# Autodesk Inventor assembly: Tetrix Honors Robotics
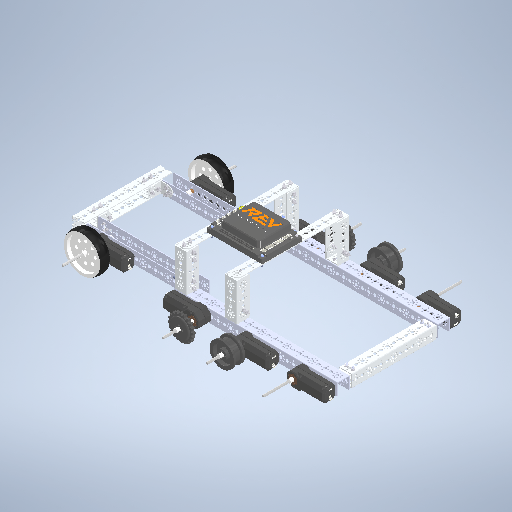
[picture p0: Inventor's stored thumbnail of the model, 512x512]
Saved by Autodesk Inventor 2025 (Build 290162010, 162A)
## iProperties
Created: 2024-11-13
Part Number: Tetrix Honors Robotics
Document SubType Name: Assembly
Designer: William Alexander
Author: William Alexander
## Documents named in this file (24)
- C:\Users\wa229389\Documents\William Alexander\Vehicles\Tetrix Honors Robotics.iam
- C:\Users\wa229389\Documents\William Alexander\Tetrix SW Parts(2)\Tetrix 416mm Channel(2)\Tetrix 416mm Channel(2).ipt
- C:\Users\wa229389\Documents\William Alexander\Tetrix SW Parts(2)\Tetrix Tank Tread Idler Wheel(2)\Tetrix Tank Tread Idler Wheel(2).ipt
- C:\Users\wa229389\Documents\William Alexander\Tetrix SW Parts(2)\Tetrix Screw 6-32 x 0.5(2)\Tetrix Screw 6-32 x 0.5(2).ipt
- C:\Users\wa229389\Documents\William Alexander\Tetrix SW Parts(2)\Tetrix Flat 288mm x26mm(2)\Tetrix Flat 288mm x26mm(2).ipt
- C:\Users\wa229389\Documents\William Alexander\Tetrix SW Parts(2)\Tetrix 96mm Channel(2)\Tetrix 96mm Channel(2).ipt
- C:\Users\wa229389\Documents\William Alexander\Tetrix SW Parts(2)\Tetrix L Bracket(2)\Tetrix L Bracket(2).ipt
- C:\Users\wa229389\Documents\William Alexander\Tetrix SW Parts(2)\Tetrix Inside C Connectors(2)\Tetrix Inside C Connectors(2).ipt
- C:\Users\wa229389\Documents\William Alexander\Tetrix SW Parts(2)\Tetrix Kep Nut(2)\Tetrix Kep Nut(2).ipt
- C:\Users\wa229389\Documents\William Alexander\Tetrix SW Parts(2)\Tetrix Tank Tread Sprocket(2)\Tetrix Tank Tread Sprocket(2).ipt
- C:\Users\wa229389\Documents\William Alexander\Tetrix SW Parts\Tetrix 416mm Channel\Tetrix 416mm Channel.ipt
- C:\Users\wa229389\Documents\William Alexander\Tetrix SW Parts\Tetrix Kep Nut\Tetrix Kep Nut.ipt
- C:\Users\wa229389\Documents\William Alexander\Tetrix SW Parts\Tetrix Screw 6-32 x 0.5\Tetrix Screw 6-32 x 0.5.ipt
- C:\Users\wa229389\Documents\William Alexander\Tetrix SW Parts\Tetrix 416mm Channel - Copy\Tetrix 416mm Channel - Copy.ipt
- C:\Users\wa229389\Documents\William Alexander\tetrix-part-library-inventor-2018-files-1.snapshot.27\Fasteners\Socket Head Cap Screws\32mm Socket Head Cap Screw.ipt
- C:\Users\wa229389\Documents\William Alexander\Tetrix SW Parts(2)\Tetrix 416mm Channel(2) - Copy\Tetrix 416mm Channel(2) - Copy.ipt
- C:\Users\wa229389\Documents\William Alexander\tetrix-part-library-inventor-2018-files-1.snapshot.27\Fasteners\Kep Nut.ipt
- C:\Users\wa229389\Documents\William Alexander\Tetrix SW Parts(2)\Tetrix Axle Spacer 0.375(2)\Tetrix Axle Spacer 0.375(2).ipt
- C:\Users\wa229389\Documents\William Alexander\rev-core-hex-motor-1.snapshot.2\REV-41-1300 (1)\REV-41-1300 (1).ipt
- C:\Users\wa229389\Documents\William Alexander\rev-core-hex-motor-1.snapshot.2\REV-41-1347\REV-41-1347.ipt
- C:\Users\wa229389\Documents\William Alexander\Tetrix SW Parts(2)\Tetrix 4 inch Wheel(2)\Tetrix 4 inch Wheel(2).ipt
- C:\Users\wa229389\Documents\William Alexander\Tetrix SW Parts(2)\Tetrix 4.7mm x 4mm L Bronze Bushing(2)\Tetrix 4.7mm x 4mm L Bronze Bushing(2).ipt
- C:\Users\wa229389\Documents\William Alexander\Tetrix SW Parts\Tetrix Ball Head Cap Screw 6-32 x 0.375\Tetrix Ball Head Cap Screw 6-32 x 0.375.ipt
- C:\Users\wa229389\Documents\William Alexander\tetrix-part-library-inventor-2018-files-1.snapshot.27\REV Expansion Hub.ipt
## Components (249 placed, 23 different names)
1. Tetrix Tank Tread Idler Wheel(2):1 — Insert:188, Insert:265
2. Tetrix Tank Tread Idler Wheel(2):2 — Insert:187, Insert:260
3. Tetrix Screw 6-32 x 0.5(2):1 — Insert:34
4. Tetrix Screw 6-32 x 0.5(2):2 — Insert:33
5. Tetrix Screw 6-32 x 0.5(2):3 — Insert:32
6. Tetrix Screw 6-32 x 0.5(2):4 — Insert:35
7. Tetrix Flat 288mm x26mm(2):1 — Mate:12, Insert:106, Insert:107, Insert:289, Mate:21, Mate:22
8. Tetrix Flat 288mm x26mm(2):2 — Mate:14, Insert:103, Insert:108, Insert:111, Insert:112, Mate:18, Insert:288
9. Tetrix 96mm Channel(2):1 — Mate:10, Insert:53, Insert:68, Insert:69, Insert:70, Insert:86, Insert:87, Insert:178
10. Tetrix 96mm Channel(2):2 — Mate:11, Insert:55, Insert:66, Insert:67, Insert:72, Insert:73, Insert:83, Insert:84, Insert:85
11. Tetrix L Bracket(2):1 — Insert:97, Mate:15, Insert:135, Insert:136, Insert:143, Insert:144, Insert:148
12. Tetrix L Bracket(2):2 — Insert:96, Insert:137, Insert:138, Insert:141, Insert:142, Insert:145, Insert:146, Insert:150
13. Tetrix Inside C Connectors(2):2 — Mate:2, Insert:2, Insert:3, Insert:4, Insert:5, Mate:6, Insert:16, Insert:17, Insert:18, Insert:19
14. Tetrix 416mm Channel(2):2 — Mate:2, Mate:3, Mate:4, Insert:6, Insert:7, Mate:5, Insert:12, Insert:13, Insert:14, Insert:15
15. Tetrix Kep Nut(2):3 — Insert:43
16. Tetrix Tank Tread Sprocket(2):1 — Insert:198, Insert:259
17. Tetrix Kep Nut(2):5 — Insert:41
18. Tetrix Kep Nut(2):6 — Insert:40
19. Tetrix Kep Nut(2):7 — Insert:42
20. Tetrix Screw 6-32 x 0.5(2):6 — Insert:3
21. Tetrix Screw 6-32 x 0.5(2):7 — Insert:2
22. Tetrix 416mm Channel:1 — Mate:6, Insert:20, Insert:21, Insert:22, Insert:23, Mate:8, Insert:32, Insert:33, Insert:34, Insert:35, Insert:52, Insert:98, Insert:202, Insert:205, Insert:211, Insert:213, Insert:215, Insert:230, Insert:231, Insert:233, Insert:276, Insert:277, Insert:278, Insert:279, Insert:280, Insert:281
23. Tetrix Kep Nut:1 — Insert:7
24. Tetrix Kep Nut:2 — Insert:6
25. Tetrix Kep Nut:3 — Mate:3
26. Tetrix Kep Nut:4 — Mate:4
27. Tetrix Screw 6-32 x 0.5:1 — Insert:5
28. Tetrix Screw 6-32 x 0.5:2 — Insert:4
29. Tetrix Screw 6-32 x 0.5:3 — Insert:9
30. Tetrix Screw 6-32 x 0.5:4 — Insert:10
31. Tetrix Screw 6-32 x 0.5:5 — Insert:11
32. Tetrix Screw 6-32 x 0.5:6 — Insert:8
33. Tetrix Inside C Connectors(2):3 — Mate:5, Insert:8, Insert:9, Insert:10, Insert:11, Mate:7, Insert:24, Insert:25, Insert:26, Insert:27
34. Tetrix Kep Nut(2):8 — Insert:15
35. Tetrix Kep Nut(2):9 — Insert:14
36. Tetrix Kep Nut(2):10 — Insert:13
37. Tetrix Kep Nut(2):11 — Insert:12
38. Tetrix Kep Nut(2):12 — Insert:22
39. Tetrix Kep Nut(2):13 — Insert:23
40. Tetrix Kep Nut(2):14 — Insert:20
41. Tetrix Kep Nut(2):15 — Insert:21
42. Tetrix 416mm Channel:2 — Mate:7, Insert:28, Insert:29, Insert:30, Insert:31, Mate:9, Insert:48, Insert:49, Insert:50, Insert:51, Insert:54, Insert:99, Insert:201, Insert:203, Insert:210, Insert:212, Insert:214, Insert:234, Insert:236, Insert:237, Insert:266, Insert:267, Insert:268, Insert:269, Insert:270, Insert:271
43. Tetrix Screw 6-32 x 0.5:7 — Insert:17
44. Tetrix Screw 6-32 x 0.5:8 — Insert:16
45. Tetrix Screw 6-32 x 0.5:9 — Insert:19
46. Tetrix Screw 6-32 x 0.5:10 — Insert:18
47. Tetrix Screw 6-32 x 0.5:11 — Insert:24
48. Tetrix Screw 6-32 x 0.5:12 — Insert:25
49. Tetrix Screw 6-32 x 0.5:13 — Insert:26
50. Tetrix Screw 6-32 x 0.5:14 — Insert:27
51. Tetrix Kep Nut:5 — Insert:29
52. Tetrix Kep Nut:6 — Insert:28
53. Tetrix Kep Nut:7 — Insert:31
54. Tetrix Kep Nut:8 — Insert:30
55. Tetrix 416mm Channel - Copy:1 — Mate:8, Insert:40, Insert:41, Insert:42, Insert:43, Insert:97, Insert:129, Insert:130, Insert:147, Insert:206, Insert:232, Insert:274, Insert:275
56. Tetrix 416mm Channel - Copy:2 — Mate:9, Insert:44, Insert:45, Insert:46, Insert:47, Insert:96, Insert:131, Insert:132, Insert:149, Insert:208, Insert:235, Insert:272, Insert:273
57. Tetrix Kep Nut:9 — Insert:45
58. Tetrix Kep Nut:10 — Insert:44
59. Tetrix Kep Nut:11 — Insert:47
60. Tetrix Kep Nut:12 — Insert:46
61. Tetrix Screw 6-32 x 0.5:15 — Insert:49
62. Tetrix Screw 6-32 x 0.5:16 — Insert:51
63. Tetrix Screw 6-32 x 0.5:17 — Insert:48
64. Tetrix Screw 6-32 x 0.5:18 — Insert:50
65. Tetrix Inside C Connectors(2):4 — Insert:53, Insert:58, Insert:60, Insert:61, Mate:19, Mate:20
66. Tetrix Inside C Connectors(2):5 — Insert:54, Mate:11, Insert:74, Insert:82, Insert:94, Insert:199
67. Tetrix Inside C Connectors(2):6 — Insert:55, Mate:12, Insert:62, Insert:63, Insert:64, Insert:65, Insert:104, Insert:105
68. Tetrix Inside C Connectors(2):7 — Insert:52, Mate:10, Insert:92, Insert:93, Insert:95, Insert:177
69. Tetrix Screw 6-32 x 0.5(2):8 — Insert:60
70. Tetrix Screw 6-32 x 0.5(2):11 — Insert:58
71. Tetrix Screw 6-32 x 0.5(2):12 — Insert:61
72. Tetrix Screw 6-32 x 0.5(2):13 — Insert:62
73. Tetrix Screw 6-32 x 0.5(2):15 — Insert:65
74. Tetrix Screw 6-32 x 0.5(2):16 — Insert:63
75. Tetrix Screw 6-32 x 0.5(2):17 — Insert:64
76. Tetrix Kep Nut(2):16 — Insert:66
77. Tetrix Kep Nut(2):17 — Insert:68
78. Tetrix Kep Nut(2):18 — Insert:69
79. Tetrix Kep Nut(2):19 — Insert:67
80. Tetrix Kep Nut(2):20 — Insert:72
81. Tetrix Kep Nut(2):21 — Insert:70
82. Tetrix Kep Nut(2):22 — Insert:73
83. Tetrix Kep Nut(2):24 — Insert:85
84. Tetrix Kep Nut(2):25 — Insert:87
85. Tetrix Kep Nut(2):26 — Insert:86
86. Tetrix Kep Nut(2):28 — Insert:83
87. Tetrix Kep Nut(2):29 — Insert:84
88. Tetrix Screw 6-32 x 0.5(2):25 — Insert:74
89. Tetrix Screw 6-32 x 0.5(2):31 — Insert:82
90. 32mm Socket Head Cap Screw:1 — Insert:92
91. 32mm Socket Head Cap Screw:2 — Insert:93
92. 32mm Socket Head Cap Screw:3 — Insert:94
93. Tetrix Screw 6-32 x 0.5(2):32 — Insert:95
94. Tetrix 96mm Channel(2):3 — Insert:101, Insert:102, Insert:171, Insert:172, Insert:185, Insert:186
95. Tetrix 96mm Channel(2):4 — Insert:100, Mate:13, Insert:175, Insert:176, Insert:181, Insert:182
96. Tetrix Inside C Connectors(2):9 — Insert:102, Insert:109, Insert:110
97. Tetrix Inside C Connectors(2):10 — Insert:99, Insert:100, Insert:173, Insert:174, Insert:179, Insert:180, Insert:200
98. Tetrix Inside C Connectors(2):11 — Insert:98, Insert:101, Insert:169, Insert:170, Insert:183, Insert:184, Insert:204
99. Tetrix Inside C Connectors(2):12 — Mate:13, Mate:14
100. Tetrix Screw 6-32 x 0.5(2):33 — Insert:103
101. Tetrix Screw 6-32 x 0.5(2):34 — Insert:105
102. Tetrix Screw 6-32 x 0.5(2):35 — Insert:104
103. Tetrix Kep Nut(2):32 — Insert:107
104. Tetrix Kep Nut(2):33 — Insert:106
105. Tetrix Kep Nut(2):34 — Insert:112
106. Tetrix Kep Nut(2):35 — Insert:111
107. Tetrix Screw 6-32 x 0.5(2):36 — Insert:109
108. Tetrix Screw 6-32 x 0.5(2):37 — Insert:110
109. Tetrix Screw 6-32 x 0.5(2):38 — Insert:108
110. Tetrix 416mm Channel(2) - Copy:1 — Insert:133, Insert:134, Mate:16, Mate:17, Insert:155, Insert:156
111. Tetrix Screw 6-32 x 0.5(2):39 — Insert:131
112. Tetrix Kep Nut(2):40 — Insert:143
113. Tetrix Kep Nut(2):41 — Insert:146
114. Tetrix Kep Nut(2):42 — Insert:144
115. Tetrix Kep Nut(2):43 — Insert:145
116. Tetrix Screw 6-32 x 0.5(2):44 — Insert:132
117. Tetrix Screw 6-32 x 0.5(2):45 — Insert:130
118. Tetrix Screw 6-32 x 0.5(2):46 — Insert:129
119. Tetrix Kep Nut(2):44 — Insert:150
120. Tetrix Kep Nut(2):45 — Mate:17
121. Tetrix Kep Nut(2):46 — Insert:138
122. Tetrix Kep Nut(2):47 — Mate:16
123. Tetrix Kep Nut(2):48 — Insert:137
124. Tetrix Kep Nut(2):49 — Insert:148
125. Tetrix Kep Nut(2):50 — Insert:136
126. Tetrix Kep Nut(2):51 — Insert:135
127. Tetrix Screw 6-32 x 0.5(2):47 — Insert:139
128. Tetrix Screw 6-32 x 0.5(2):48 — Insert:141
129. Tetrix Screw 6-32 x 0.5(2):49 — Insert:142
130. Tetrix Screw 6-32 x 0.5(2):50 — Insert:140
131. Tetrix Screw 6-32 x 0.5(2):51 — Insert:151
132. Tetrix Screw 6-32 x 0.5(2):52 — Insert:152
133. Tetrix Screw 6-32 x 0.5(2):53 — Insert:149
134. Tetrix Screw 6-32 x 0.5(2):54 — Insert:147
135. Tetrix Inside C Connectors(2):13 — Mate:15, Insert:133, Insert:139, Insert:140, Insert:151, Insert:152
136. Tetrix Inside C Connectors(2):14 — Insert:134, Insert:153, Insert:154
137. Tetrix Screw 6-32 x 0.5(2):55 — Insert:153
138. Tetrix Screw 6-32 x 0.5(2):56 — Insert:154
139. Tetrix Kep Nut(2):52 — Insert:156
140. Tetrix Kep Nut(2):53 — Insert:155
141. Tetrix Kep Nut(2):54 — Insert:176
142. Tetrix Kep Nut(2):55 — Insert:175
143. Tetrix Kep Nut(2):56 — Insert:182
144. Tetrix Kep Nut(2):57 — Insert:181
145. Tetrix Kep Nut(2):58 — Insert:172
146. Tetrix Kep Nut(2):59 — Insert:171
147. Tetrix Kep Nut(2):61 — Insert:178
148. Tetrix Screw 6-32 x 0.5(2):57 — Insert:170
149. Tetrix Screw 6-32 x 0.5(2):58 — Insert:169
150. Tetrix Screw 6-32 x 0.5(2):59 — Insert:174
151. Tetrix Screw 6-32 x 0.5(2):60 — Insert:173
152. Tetrix Screw 6-32 x 0.5(2):61 — Insert:184
153. Tetrix Screw 6-32 x 0.5(2):62 — Insert:183
154. Tetrix Screw 6-32 x 0.5(2):63 — Insert:180
155. Tetrix Screw 6-32 x 0.5(2):64 — Insert:179
156. 32mm Socket Head Cap Screw:4 — Insert:177
157. Tetrix Kep Nut(2):62 — Insert:185
158. Tetrix Kep Nut(2):63 — Insert:186
159. Tetrix Axle Spacer 0.375(2):2 — Insert:188
160. Tetrix Axle Spacer 0.375(2):3 — Insert:187
161. REV-41-1300 (1):1 — Insert:230, Insert:255
162. REV-41-1300 (1):2 — Insert:231, Insert:256
163. REV-41-1300 (1):3 — Insert:235, Insert:254
164. REV-41-1300 (1):4 — Insert:232, Insert:257
165. REV-41-1300 (1):5 — Insert:234, Insert:251
166. REV-41-1300 (1):6 — Insert:233, Insert:238
167. REV-41-1300 (1):7 — Insert:236, Insert:252
168. REV-41-1300 (1):8 — Insert:237, Insert:253
169. Tetrix Axle Spacer 0.375(2):7 — Insert:198, Insert:258
170. Tetrix Screw 6-32 x 0.5(2):65 — Insert:204
171. Tetrix Screw 6-32 x 0.5(2):66 — Insert:199
172. Tetrix Screw 6-32 x 0.5(2):67 — Insert:200
173. Tetrix Kep Nut(2):64 — Insert:205
174. Tetrix Kep Nut(2):65 — Insert:202
175. Tetrix Kep Nut(2):66 — Insert:203
176. Tetrix Kep Nut(2):67 — Insert:201
177. Tetrix 4 inch Wheel(2):1 — Insert:261, Insert:263
178. Tetrix 4 inch Wheel(2):2 — Insert:262, Insert:264
179. Tetrix 4.7mm x 4mm L Bronze Bushing(2):1 — Insert:215, Insert:219
180. Tetrix 4.7mm x 4mm L Bronze Bushing(2):2 — Insert:214, Insert:216
181. Tetrix 4.7mm x 4mm L Bronze Bushing(2):3 — Insert:213, Insert:220
182. Tetrix 4.7mm x 4mm L Bronze Bushing(2):4 — Insert:212, Insert:217
183. Tetrix 4.7mm x 4mm L Bronze Bushing(2):5 — Insert:211, Insert:221
184. Tetrix 4.7mm x 4mm L Bronze Bushing(2):6 — Insert:210, Insert:218
185. Tetrix 4.7mm x 4mm L Bronze Bushing(2):7 — Insert:208, Insert:209
186. Tetrix 4.7mm x 4mm L Bronze Bushing(2):8 — Insert:206, Insert:207
187. REV-41-1347:11 — Insert:225
188. REV-41-1347:12 — Insert:226
189. REV-41-1347:13 — Insert:228
190. REV-41-1347:14 — Insert:229
191. REV-41-1347:15 — Insert:227
192. REV-41-1347:16 — Insert:224
193. REV-41-1347:17 — Insert:223
194. REV-41-1347:18 — Insert:222
195. Tetrix Axle Spacer 0.375(2):8 — Insert:221, Insert:229
196. Tetrix Axle Spacer 0.375(2):9 — Insert:220, Insert:228
197. Tetrix Axle Spacer 0.375(2):10 — Insert:219, Insert:227
198. Tetrix Axle Spacer 0.375(2):11 — Insert:218, Insert:226
199. Tetrix Axle Spacer 0.375(2):12 — Insert:217, Insert:225
200. Tetrix Axle Spacer 0.375(2):13 — Insert:216, Insert:224
201. Tetrix Axle Spacer 0.375(2):14 — Insert:209, Insert:222
202. Tetrix Axle Spacer 0.375(2):15 — Insert:207, Insert:223
203. Tetrix Axle Spacer 0.375(2):16 — Insert:259
204. Tetrix Axle Spacer 0.375(2):17 — Insert:262
205. Tetrix Axle Spacer 0.375(2):18 — Insert:261
206. Tetrix Axle Spacer 0.375(2):19 — Insert:257, Insert:263
207. Tetrix Axle Spacer 0.375(2):20 — Insert:256, Insert:260
208. Tetrix Axle Spacer 0.375(2):21 — Insert:253
209. Tetrix Axle Spacer 0.375(2):23 — Insert:238, Insert:239
210. Tetrix Axle Spacer 0.375(2):24 — Insert:251, Insert:258
211. Tetrix Axle Spacer 0.375(2):25 — Insert:252, Insert:265
212. Tetrix Axle Spacer 0.375(2):26 — Insert:254, Insert:264
213. Tetrix Axle Spacer 0.375(2):27 — Insert:255
214. Tetrix Tank Tread Sprocket(2):3 — Insert:240, Insert:241, Insert:245, Insert:246, Insert:247, Insert:248, Insert:249, Insert:250
215. Tetrix Axle Spacer 0.375(2):32 — Insert:241
216. Tetrix Axle Spacer 0.375(2):33 — Insert:239, Insert:240
217. Kep Nut:7 — Insert:245
218. Kep Nut:8 — Insert:247
219. Kep Nut:9 — Insert:246
220. 32mm Socket Head Cap Screw:5 — Insert:248
221. 32mm Socket Head Cap Screw:6 — Insert:249
222. 32mm Socket Head Cap Screw:7 — Insert:250
223. Tetrix Ball Head Cap Screw 6-32 x 0.375:1 — Insert:267
224. Tetrix Ball Head Cap Screw 6-32 x 0.375:2 — Insert:266
225. Tetrix Ball Head Cap Screw 6-32 x 0.375:3 — Insert:268
226. Tetrix Ball Head Cap Screw 6-32 x 0.375:4 — Insert:269
227. Tetrix Ball Head Cap Screw 6-32 x 0.375:5 — Insert:270
228. Tetrix Ball Head Cap Screw 6-32 x 0.375:6 — Insert:271
229. Tetrix Ball Head Cap Screw 6-32 x 0.375:7 — Insert:273
230. Tetrix Ball Head Cap Screw 6-32 x 0.375:8 — Insert:272
231. Tetrix Ball Head Cap Screw 6-32 x 0.375:9 — Insert:277
232. Tetrix Ball Head Cap Screw 6-32 x 0.375:10 — Insert:276
233. Tetrix Ball Head Cap Screw 6-32 x 0.375:11 — Insert:275
234. Tetrix Ball Head Cap Screw 6-32 x 0.375:12 — Insert:274
235. Tetrix Ball Head Cap Screw 6-32 x 0.375:13 — Insert:278
236. Tetrix Ball Head Cap Screw 6-32 x 0.375:14 — Insert:279
237. Tetrix Ball Head Cap Screw 6-32 x 0.375:15 — Insert:281
238. Tetrix Ball Head Cap Screw 6-32 x 0.375:16 — Insert:280
239. REV Expansion Hub:1 — Insert:283, Insert:285, Mate:18, Insert:286, Insert:287
240. Tetrix Kep Nut(2):70 — Insert:288
241. Tetrix Kep Nut(2):71 — Insert:289
242. 32mm Socket Head Cap Screw:9 — Insert:285
243. 32mm Socket Head Cap Screw:10 — Insert:283
244. Tetrix Screw 6-32 x 0.5(2):68 — Insert:287
245. Tetrix Screw 6-32 x 0.5(2):69 — Insert:286
246. Tetrix Kep Nut(2):72 — Mate:21
247. Tetrix Kep Nut(2):73 — Mate:22
248. Tetrix Screw 6-32 x 0.5(2):70 — Mate:19
249. Tetrix Screw 6-32 x 0.5(2):71 — Mate:20
## Relationships (248: Insert 227, Mate 21)
- Mate:2: Tetrix Inside C Connectors(2):2 ↔ Tetrix 416mm Channel(2):2
- Insert:2: Tetrix Inside C Connectors(2):2 ↔ Tetrix Screw 6-32 x 0.5(2):7
- Insert:3: Tetrix Inside C Connectors(2):2 ↔ Tetrix Screw 6-32 x 0.5(2):6
- Mate:3: Tetrix 416mm Channel(2):2 ↔ Tetrix Kep Nut:3
- Mate:4: Tetrix 416mm Channel(2):2 ↔ Tetrix Kep Nut:4
- Insert:4: Tetrix Inside C Connectors(2):2 ↔ Tetrix Screw 6-32 x 0.5:2
- Insert:5: Tetrix Inside C Connectors(2):2 ↔ Tetrix Screw 6-32 x 0.5:1
- Insert:6: Tetrix 416mm Channel(2):2 ↔ Tetrix Kep Nut:2
- Insert:7: Tetrix 416mm Channel(2):2 ↔ Tetrix Kep Nut:1
- Mate:5: Tetrix 416mm Channel(2):2 ↔ Tetrix Inside C Connectors(2):3
- Insert:8: Tetrix Screw 6-32 x 0.5:6 ↔ Tetrix Inside C Connectors(2):3
- Insert:9: Tetrix Screw 6-32 x 0.5:3 ↔ Tetrix Inside C Connectors(2):3
- Insert:10: Tetrix Screw 6-32 x 0.5:4 ↔ Tetrix Inside C Connectors(2):3
- Insert:11: Tetrix Screw 6-32 x 0.5:5 ↔ Tetrix Inside C Connectors(2):3
- Insert:12: Tetrix 416mm Channel(2):2 ↔ Tetrix Kep Nut(2):11
- Insert:13: Tetrix 416mm Channel(2):2 ↔ Tetrix Kep Nut(2):10
- Insert:14: Tetrix 416mm Channel(2):2 ↔ Tetrix Kep Nut(2):9
- Insert:15: Tetrix 416mm Channel(2):2 ↔ Tetrix Kep Nut(2):8
- Mate:6: Tetrix Inside C Connectors(2):2 ↔ Tetrix 416mm Channel:1
- Mate:7: Tetrix Inside C Connectors(2):3 ↔ Tetrix 416mm Channel:2
- Insert:16: Tetrix Inside C Connectors(2):2 ↔ Tetrix Screw 6-32 x 0.5:8
- Insert:17: Tetrix Inside C Connectors(2):2 ↔ Tetrix Screw 6-32 x 0.5:7
- Insert:18: Tetrix Inside C Connectors(2):2 ↔ Tetrix Screw 6-32 x 0.5:10
- Insert:19: Tetrix Inside C Connectors(2):2 ↔ Tetrix Screw 6-32 x 0.5:9
- Insert:20: Tetrix 416mm Channel:1 ↔ Tetrix Kep Nut(2):14
- Insert:21: Tetrix 416mm Channel:1 ↔ Tetrix Kep Nut(2):15
- Insert:22: Tetrix 416mm Channel:1 ↔ Tetrix Kep Nut(2):12
- Insert:23: Tetrix 416mm Channel:1 ↔ Tetrix Kep Nut(2):13
- Insert:24: Tetrix Inside C Connectors(2):3 ↔ Tetrix Screw 6-32 x 0.5:11
- Insert:25: Tetrix Inside C Connectors(2):3 ↔ Tetrix Screw 6-32 x 0.5:12
- Insert:26: Tetrix Inside C Connectors(2):3 ↔ Tetrix Screw 6-32 x 0.5:13
- Insert:27: Tetrix Inside C Connectors(2):3 ↔ Tetrix Screw 6-32 x 0.5:14
- Insert:28: Tetrix 416mm Channel:2 ↔ Tetrix Kep Nut:6
- Insert:29: Tetrix 416mm Channel:2 ↔ Tetrix Kep Nut:5
- Insert:30: Tetrix 416mm Channel:2 ↔ Tetrix Kep Nut:8
- Insert:31: Tetrix 416mm Channel:2 ↔ Tetrix Kep Nut:7
- Mate:8: Tetrix 416mm Channel:1 ↔ Tetrix 416mm Channel - Copy:1
- Mate:9: Tetrix 416mm Channel:2 ↔ Tetrix 416mm Channel - Copy:2
- Insert:32: Tetrix Screw 6-32 x 0.5(2):3 ↔ Tetrix 416mm Channel:1
- Insert:33: Tetrix Screw 6-32 x 0.5(2):2 ↔ Tetrix 416mm Channel:1
- Insert:34: Tetrix Screw 6-32 x 0.5(2):1 ↔ Tetrix 416mm Channel:1
- Insert:35: Tetrix Screw 6-32 x 0.5(2):4 ↔ Tetrix 416mm Channel:1
- Insert:40: Tetrix Kep Nut(2):6 ↔ Tetrix 416mm Channel - Copy:1
- Insert:41: Tetrix Kep Nut(2):5 ↔ Tetrix 416mm Channel - Copy:1
- Insert:42: Tetrix Kep Nut(2):7 ↔ Tetrix 416mm Channel - Copy:1
- Insert:43: Tetrix Kep Nut(2):3 ↔ Tetrix 416mm Channel - Copy:1
- Insert:44: Tetrix 416mm Channel - Copy:2 ↔ Tetrix Kep Nut:10
- Insert:45: Tetrix 416mm Channel - Copy:2 ↔ Tetrix Kep Nut:9
- Insert:46: Tetrix 416mm Channel - Copy:2 ↔ Tetrix Kep Nut:12
- Insert:47: Tetrix 416mm Channel - Copy:2 ↔ Tetrix Kep Nut:11
- Insert:48: Tetrix 416mm Channel:2 ↔ Tetrix Screw 6-32 x 0.5:17
- Insert:49: Tetrix 416mm Channel:2 ↔ Tetrix Screw 6-32 x 0.5:15
- Insert:50: Tetrix 416mm Channel:2 ↔ Tetrix Screw 6-32 x 0.5:18
- Insert:51: Tetrix 416mm Channel:2 ↔ Tetrix Screw 6-32 x 0.5:16
- Insert:52: Tetrix 416mm Channel:1 ↔ Tetrix Inside C Connectors(2):7
- Mate:10: Tetrix 96mm Channel(2):1 ↔ Tetrix Inside C Connectors(2):7
- Insert:53: Tetrix 96mm Channel(2):1 ↔ Tetrix Inside C Connectors(2):4
- Insert:54: Tetrix 416mm Channel:2 ↔ Tetrix Inside C Connectors(2):5
- Mate:11: Tetrix 96mm Channel(2):2 ↔ Tetrix Inside C Connectors(2):5
- Insert:55: Tetrix 96mm Channel(2):2 ↔ Tetrix Inside C Connectors(2):6
- Mate:12: Tetrix Flat 288mm x26mm(2):1 ↔ Tetrix Inside C Connectors(2):6
- Insert:58: Tetrix Inside C Connectors(2):4 ↔ Tetrix Screw 6-32 x 0.5(2):11
- Insert:60: Tetrix Inside C Connectors(2):4 ↔ Tetrix Screw 6-32 x 0.5(2):8
- Insert:61: Tetrix Inside C Connectors(2):4 ↔ Tetrix Screw 6-32 x 0.5(2):12
- Insert:62: Tetrix Inside C Connectors(2):6 ↔ Tetrix Screw 6-32 x 0.5(2):13
- Insert:63: Tetrix Inside C Connectors(2):6 ↔ Tetrix Screw 6-32 x 0.5(2):16
- Insert:64: Tetrix Inside C Connectors(2):6 ↔ Tetrix Screw 6-32 x 0.5(2):17
- Insert:65: Tetrix Inside C Connectors(2):6 ↔ Tetrix Screw 6-32 x 0.5(2):15
- Insert:66: Tetrix 96mm Channel(2):2 ↔ Tetrix Kep Nut(2):16
- Insert:67: Tetrix 96mm Channel(2):2 ↔ Tetrix Kep Nut(2):19
- Insert:68: Tetrix 96mm Channel(2):1 ↔ Tetrix Kep Nut(2):17
- Insert:69: Tetrix 96mm Channel(2):1 ↔ Tetrix Kep Nut(2):18
- Insert:70: Tetrix 96mm Channel(2):1 ↔ Tetrix Kep Nut(2):21
- Insert:72: Tetrix 96mm Channel(2):2 ↔ Tetrix Kep Nut(2):20
- Insert:73: Tetrix 96mm Channel(2):2 ↔ Tetrix Kep Nut(2):22
- Insert:74: Tetrix Inside C Connectors(2):5 ↔ Tetrix Screw 6-32 x 0.5(2):25
- Insert:82: Tetrix Inside C Connectors(2):5 ↔ Tetrix Screw 6-32 x 0.5(2):31
- Insert:83: Tetrix 96mm Channel(2):2 ↔ Tetrix Kep Nut(2):28
- Insert:84: Tetrix 96mm Channel(2):2 ↔ Tetrix Kep Nut(2):29
- Insert:85: Tetrix 96mm Channel(2):2 ↔ Tetrix Kep Nut(2):24
- Insert:86: Tetrix 96mm Channel(2):1 ↔ Tetrix Kep Nut(2):26
- Insert:87: Tetrix 96mm Channel(2):1 ↔ Tetrix Kep Nut(2):25
- Insert:92: Tetrix Inside C Connectors(2):7 ↔ 32mm Socket Head Cap Screw:1
- Insert:93: Tetrix Inside C Connectors(2):7 ↔ 32mm Socket Head Cap Screw:2
- Insert:94: Tetrix Inside C Connectors(2):5 ↔ 32mm Socket Head Cap Screw:3
- Insert:95: Tetrix Inside C Connectors(2):7 ↔ Tetrix Screw 6-32 x 0.5(2):32
- Insert:96: Tetrix L Bracket(2):2 ↔ Tetrix 416mm Channel - Copy:2
- Insert:97: Tetrix L Bracket(2):1 ↔ Tetrix 416mm Channel - Copy:1
- Insert:98: Tetrix 416mm Channel:1 ↔ Tetrix Inside C Connectors(2):11
- Insert:99: Tetrix 416mm Channel:2 ↔ Tetrix Inside C Connectors(2):10
- Insert:100: Tetrix 96mm Channel(2):4 ↔ Tetrix Inside C Connectors(2):10
- Insert:101: Tetrix 96mm Channel(2):3 ↔ Tetrix Inside C Connectors(2):11
- Insert:102: Tetrix 96mm Channel(2):3 ↔ Tetrix Inside C Connectors(2):9
- Mate:13: Tetrix 96mm Channel(2):4 ↔ Tetrix Inside C Connectors(2):12
- Mate:14: Tetrix Flat 288mm x26mm(2):2 ↔ Tetrix Inside C Connectors(2):12
- Insert:103: Tetrix Flat 288mm x26mm(2):2 ↔ Tetrix Screw 6-32 x 0.5(2):33
- Insert:104: Tetrix Inside C Connectors(2):6 ↔ Tetrix Screw 6-32 x 0.5(2):35
- Insert:105: Tetrix Inside C Connectors(2):6 ↔ Tetrix Screw 6-32 x 0.5(2):34
- Insert:106: Tetrix Flat 288mm x26mm(2):1 ↔ Tetrix Kep Nut(2):33
- Insert:107: Tetrix Flat 288mm x26mm(2):1 ↔ Tetrix Kep Nut(2):32
- Insert:108: Tetrix Flat 288mm x26mm(2):2 ↔ Tetrix Screw 6-32 x 0.5(2):38
- Insert:109: Tetrix Inside C Connectors(2):9 ↔ Tetrix Screw 6-32 x 0.5(2):36
- Insert:110: Tetrix Inside C Connectors(2):9 ↔ Tetrix Screw 6-32 x 0.5(2):37
- Insert:111: Tetrix Flat 288mm x26mm(2):2 ↔ Tetrix Kep Nut(2):35
- Insert:112: Tetrix Flat 288mm x26mm(2):2 ↔ Tetrix Kep Nut(2):34
- Insert:129: Tetrix 416mm Channel - Copy:1 ↔ Tetrix Screw 6-32 x 0.5(2):46
- Insert:130: Tetrix 416mm Channel - Copy:1 ↔ Tetrix Screw 6-32 x 0.5(2):45
- Insert:131: Tetrix 416mm Channel - Copy:2 ↔ Tetrix Screw 6-32 x 0.5(2):39
- Insert:132: Tetrix 416mm Channel - Copy:2 ↔ Tetrix Screw 6-32 x 0.5(2):44
- Mate:15: Tetrix L Bracket(2):1 ↔ Tetrix Inside C Connectors(2):13
- Insert:133: Tetrix 416mm Channel(2) - Copy:1 ↔ Tetrix Inside C Connectors(2):13
- Insert:134: Tetrix 416mm Channel(2) - Copy:1 ↔ Tetrix Inside C Connectors(2):14
- Insert:135: Tetrix L Bracket(2):1 ↔ Tetrix Kep Nut(2):51
- Insert:136: Tetrix L Bracket(2):1 ↔ Tetrix Kep Nut(2):50
- Insert:137: Tetrix L Bracket(2):2 ↔ Tetrix Kep Nut(2):48
- Insert:138: Tetrix L Bracket(2):2 ↔ Tetrix Kep Nut(2):46
- Insert:139: Tetrix Screw 6-32 x 0.5(2):47 ↔ Tetrix Inside C Connectors(2):13
- Insert:140: Tetrix Screw 6-32 x 0.5(2):50 ↔ Tetrix Inside C Connectors(2):13
- Insert:141 (2.54 mm): Tetrix L Bracket(2):2 ↔ Tetrix Screw 6-32 x 0.5(2):48
- Insert:142 (2.54 mm): Tetrix L Bracket(2):2 ↔ Tetrix Screw 6-32 x 0.5(2):49
- Insert:143: Tetrix L Bracket(2):1 ↔ Tetrix Kep Nut(2):40
- Insert:144: Tetrix L Bracket(2):1 ↔ Tetrix Kep Nut(2):42
- Insert:145: Tetrix L Bracket(2):2 ↔ Tetrix Kep Nut(2):43
- Insert:146: Tetrix L Bracket(2):2 ↔ Tetrix Kep Nut(2):41
- Insert:147: Tetrix 416mm Channel - Copy:1 ↔ Tetrix Screw 6-32 x 0.5(2):54
- Insert:148: Tetrix L Bracket(2):1 ↔ Tetrix Kep Nut(2):49
- Insert:149: Tetrix 416mm Channel - Copy:2 ↔ Tetrix Screw 6-32 x 0.5(2):53
- Insert:150: Tetrix L Bracket(2):2 ↔ Tetrix Kep Nut(2):44
- Insert:151: Tetrix Screw 6-32 x 0.5(2):51 ↔ Tetrix Inside C Connectors(2):13
- Insert:152: Tetrix Screw 6-32 x 0.5(2):52 ↔ Tetrix Inside C Connectors(2):13
- Insert:153: Tetrix Inside C Connectors(2):14 ↔ Tetrix Screw 6-32 x 0.5(2):55
- Insert:154: Tetrix Inside C Connectors(2):14 ↔ Tetrix Screw 6-32 x 0.5(2):56
- Mate:16: Tetrix 416mm Channel(2) - Copy:1 ↔ Tetrix Kep Nut(2):47
- Mate:17: Tetrix 416mm Channel(2) - Copy:1 ↔ Tetrix Kep Nut(2):45
- Insert:155: Tetrix 416mm Channel(2) - Copy:1 ↔ Tetrix Kep Nut(2):53
- Insert:156: Tetrix 416mm Channel(2) - Copy:1 ↔ Tetrix Kep Nut(2):52
- Insert:169: Tetrix Inside C Connectors(2):11 ↔ Tetrix Screw 6-32 x 0.5(2):58
- Insert:170: Tetrix Inside C Connectors(2):11 ↔ Tetrix Screw 6-32 x 0.5(2):57
- Insert:171: Tetrix 96mm Channel(2):3 ↔ Tetrix Kep Nut(2):59
- Insert:172: Tetrix 96mm Channel(2):3 ↔ Tetrix Kep Nut(2):58
- Insert:173: Tetrix Inside C Connectors(2):10 ↔ Tetrix Screw 6-32 x 0.5(2):60
- Insert:174: Tetrix Inside C Connectors(2):10 ↔ Tetrix Screw 6-32 x 0.5(2):59
- Insert:175: Tetrix 96mm Channel(2):4 ↔ Tetrix Kep Nut(2):55
- Insert:176: Tetrix 96mm Channel(2):4 ↔ Tetrix Kep Nut(2):54
- Insert:177: Tetrix Inside C Connectors(2):7 ↔ 32mm Socket Head Cap Screw:4
- Insert:178: Tetrix 96mm Channel(2):1 ↔ Tetrix Kep Nut(2):61
- Insert:179: Tetrix Inside C Connectors(2):10 ↔ Tetrix Screw 6-32 x 0.5(2):64
- Insert:180: Tetrix Inside C Connectors(2):10 ↔ Tetrix Screw 6-32 x 0.5(2):63
- Insert:181: Tetrix 96mm Channel(2):4 ↔ Tetrix Kep Nut(2):57
- Insert:182: Tetrix 96mm Channel(2):4 ↔ Tetrix Kep Nut(2):56
- Insert:183: Tetrix Inside C Connectors(2):11 ↔ Tetrix Screw 6-32 x 0.5(2):62
- Insert:184: Tetrix Inside C Connectors(2):11 ↔ Tetrix Screw 6-32 x 0.5(2):61
- Insert:185: Tetrix 96mm Channel(2):3 ↔ Tetrix Kep Nut(2):62
- Insert:186: Tetrix 96mm Channel(2):3 ↔ Tetrix Kep Nut(2):63
- Insert:187: Tetrix Tank Tread Idler Wheel(2):2 ↔ Tetrix Axle Spacer 0.375(2):3
- Insert:188: Tetrix Tank Tread Idler Wheel(2):1 ↔ Tetrix Axle Spacer 0.375(2):2
- Insert:198: Tetrix Tank Tread Sprocket(2):1 ↔ Tetrix Axle Spacer 0.375(2):7
- Insert:199: Tetrix Inside C Connectors(2):5 ↔ Tetrix Screw 6-32 x 0.5(2):66
- Insert:200: Tetrix Inside C Connectors(2):10 ↔ Tetrix Screw 6-32 x 0.5(2):67
- Insert:201: Tetrix 416mm Channel:2 ↔ Tetrix Kep Nut(2):67
- Insert:202: Tetrix 416mm Channel:1 ↔ Tetrix Kep Nut(2):65
- Insert:203: Tetrix 416mm Channel:2 ↔ Tetrix Kep Nut(2):66
- Insert:204: Tetrix Inside C Connectors(2):11 ↔ Tetrix Screw 6-32 x 0.5(2):65
- Insert:205: Tetrix 416mm Channel:1 ↔ Tetrix Kep Nut(2):64
- Insert:206: Tetrix 416mm Channel - Copy:1 ↔ Tetrix 4.7mm x 4mm L Bronze Bushing(2):8
- Insert:207: Tetrix 4.7mm x 4mm L Bronze Bushing(2):8 ↔ Tetrix Axle Spacer 0.375(2):15
- Insert:208: Tetrix 416mm Channel - Copy:2 ↔ Tetrix 4.7mm x 4mm L Bronze Bushing(2):7
- Insert:209: Tetrix 4.7mm x 4mm L Bronze Bushing(2):7 ↔ Tetrix Axle Spacer 0.375(2):14
- Insert:210: Tetrix 416mm Channel:2 ↔ Tetrix 4.7mm x 4mm L Bronze Bushing(2):6
- Insert:211: Tetrix 416mm Channel:1 ↔ Tetrix 4.7mm x 4mm L Bronze Bushing(2):5
- Insert:212: Tetrix 416mm Channel:2 ↔ Tetrix 4.7mm x 4mm L Bronze Bushing(2):4
- Insert:213: Tetrix 416mm Channel:1 ↔ Tetrix 4.7mm x 4mm L Bronze Bushing(2):3
- Insert:214: Tetrix 416mm Channel:2 ↔ Tetrix 4.7mm x 4mm L Bronze Bushing(2):2
- Insert:215: Tetrix 416mm Channel:1 ↔ Tetrix 4.7mm x 4mm L Bronze Bushing(2):1
- Insert:216: Tetrix 4.7mm x 4mm L Bronze Bushing(2):2 ↔ Tetrix Axle Spacer 0.375(2):13
- Insert:217: Tetrix 4.7mm x 4mm L Bronze Bushing(2):4 ↔ Tetrix Axle Spacer 0.375(2):12
- Insert:218: Tetrix 4.7mm x 4mm L Bronze Bushing(2):6 ↔ Tetrix Axle Spacer 0.375(2):11
- Insert:219: Tetrix 4.7mm x 4mm L Bronze Bushing(2):1 ↔ Tetrix Axle Spacer 0.375(2):10
- Insert:220: Tetrix 4.7mm x 4mm L Bronze Bushing(2):3 ↔ Tetrix Axle Spacer 0.375(2):9
- Insert:221: Tetrix 4.7mm x 4mm L Bronze Bushing(2):5 ↔ Tetrix Axle Spacer 0.375(2):8
- Insert:222: REV-41-1347:18 ↔ Tetrix Axle Spacer 0.375(2):14
- Insert:223: REV-41-1347:17 ↔ Tetrix Axle Spacer 0.375(2):15
- Insert:224: REV-41-1347:16 ↔ Tetrix Axle Spacer 0.375(2):13
- Insert:225: REV-41-1347:11 ↔ Tetrix Axle Spacer 0.375(2):12
- Insert:226: REV-41-1347:12 ↔ Tetrix Axle Spacer 0.375(2):11
- Insert:227: REV-41-1347:15 ↔ Tetrix Axle Spacer 0.375(2):10
- Insert:228: REV-41-1347:13 ↔ Tetrix Axle Spacer 0.375(2):9
- Insert:229: REV-41-1347:14 ↔ Tetrix Axle Spacer 0.375(2):8
- Insert:230: Tetrix 416mm Channel:1 ↔ REV-41-1300 (1):1
- Insert:231: Tetrix 416mm Channel:1 ↔ REV-41-1300 (1):2
- Insert:232: Tetrix 416mm Channel - Copy:1 ↔ REV-41-1300 (1):4
- Insert:233: Tetrix 416mm Channel:1 ↔ REV-41-1300 (1):6
- Insert:234: Tetrix 416mm Channel:2 ↔ REV-41-1300 (1):5
- Insert:235: Tetrix 416mm Channel - Copy:2 ↔ REV-41-1300 (1):3
- Insert:236: Tetrix 416mm Channel:2 ↔ REV-41-1300 (1):7
- Insert:237: Tetrix 416mm Channel:2 ↔ REV-41-1300 (1):8
- Insert:238: REV-41-1300 (1):6 ↔ Tetrix Axle Spacer 0.375(2):23
- Insert:239: Tetrix Axle Spacer 0.375(2):23 ↔ Tetrix Axle Spacer 0.375(2):33
- Insert:240: Tetrix Tank Tread Sprocket(2):3 ↔ Tetrix Axle Spacer 0.375(2):33
- Insert:241: Tetrix Tank Tread Sprocket(2):3 ↔ Tetrix Axle Spacer 0.375(2):32
- Insert:245: Tetrix Tank Tread Sprocket(2):3 ↔ Kep Nut:7
- Insert:246: Tetrix Tank Tread Sprocket(2):3 ↔ Kep Nut:9
- Insert:247: Tetrix Tank Tread Sprocket(2):3 ↔ Kep Nut:8
- Insert:248: Tetrix Tank Tread Sprocket(2):3 ↔ 32mm Socket Head Cap Screw:5
- Insert:249: Tetrix Tank Tread Sprocket(2):3 ↔ 32mm Socket Head Cap Screw:6
- Insert:250: Tetrix Tank Tread Sprocket(2):3 ↔ 32mm Socket Head Cap Screw:7
- Insert:251: REV-41-1300 (1):5 ↔ Tetrix Axle Spacer 0.375(2):24
- Insert:252: REV-41-1300 (1):7 ↔ Tetrix Axle Spacer 0.375(2):25
- Insert:253: REV-41-1300 (1):8 ↔ Tetrix Axle Spacer 0.375(2):21
- Insert:254: REV-41-1300 (1):3 ↔ Tetrix Axle Spacer 0.375(2):26
- Insert:255: REV-41-1300 (1):1 ↔ Tetrix Axle Spacer 0.375(2):27
- Insert:256: REV-41-1300 (1):2 ↔ Tetrix Axle Spacer 0.375(2):20
- Insert:257: REV-41-1300 (1):4 ↔ Tetrix Axle Spacer 0.375(2):19
- Insert:258: Tetrix Axle Spacer 0.375(2):7 ↔ Tetrix Axle Spacer 0.375(2):24
- Insert:259: Tetrix Tank Tread Sprocket(2):1 ↔ Tetrix Axle Spacer 0.375(2):16
- Insert:260: Tetrix Tank Tread Idler Wheel(2):2 ↔ Tetrix Axle Spacer 0.375(2):20
- Insert:261: Tetrix 4 inch Wheel(2):1 ↔ Tetrix Axle Spacer 0.375(2):18
- Insert:262: Tetrix 4 inch Wheel(2):2 ↔ Tetrix Axle Spacer 0.375(2):17
- Insert:263: Tetrix 4 inch Wheel(2):1 ↔ Tetrix Axle Spacer 0.375(2):19
- Insert:264: Tetrix 4 inch Wheel(2):2 ↔ Tetrix Axle Spacer 0.375(2):26
- Insert:265: Tetrix Tank Tread Idler Wheel(2):1 ↔ Tetrix Axle Spacer 0.375(2):25
- Insert:266: Tetrix 416mm Channel:2 ↔ Tetrix Ball Head Cap Screw 6-32 x 0.375:2
- Insert:267: Tetrix 416mm Channel:2 ↔ Tetrix Ball Head Cap Screw 6-32 x 0.375:1
- Insert:268: Tetrix 416mm Channel:2 ↔ Tetrix Ball Head Cap Screw 6-32 x 0.375:3
- Insert:269: Tetrix 416mm Channel:2 ↔ Tetrix Ball Head Cap Screw 6-32 x 0.375:4
- Insert:270: Tetrix 416mm Channel:2 ↔ Tetrix Ball Head Cap Screw 6-32 x 0.375:5
- Insert:271: Tetrix 416mm Channel:2 ↔ Tetrix Ball Head Cap Screw 6-32 x 0.375:6
- Insert:272: Tetrix 416mm Channel - Copy:2 ↔ Tetrix Ball Head Cap Screw 6-32 x 0.375:8
- Insert:273: Tetrix 416mm Channel - Copy:2 ↔ Tetrix Ball Head Cap Screw 6-32 x 0.375:7
- Insert:274: Tetrix 416mm Channel - Copy:1 ↔ Tetrix Ball Head Cap Screw 6-32 x 0.375:12
- Insert:275: Tetrix 416mm Channel - Copy:1 ↔ Tetrix Ball Head Cap Screw 6-32 x 0.375:11
- Insert:276: Tetrix 416mm Channel:1 ↔ Tetrix Ball Head Cap Screw 6-32 x 0.375:10
- Insert:277: Tetrix 416mm Channel:1 ↔ Tetrix Ball Head Cap Screw 6-32 x 0.375:9
- Insert:278: Tetrix 416mm Channel:1 ↔ Tetrix Ball Head Cap Screw 6-32 x 0.375:13
- Insert:279: Tetrix 416mm Channel:1 ↔ Tetrix Ball Head Cap Screw 6-32 x 0.375:14
- Insert:280: Tetrix 416mm Channel:1 ↔ Tetrix Ball Head Cap Screw 6-32 x 0.375:16
- Insert:281: Tetrix 416mm Channel:1 ↔ Tetrix Ball Head Cap Screw 6-32 x 0.375:15
- Insert:283: REV Expansion Hub:1 ↔ 32mm Socket Head Cap Screw:10
- Insert:285: REV Expansion Hub:1 ↔ 32mm Socket Head Cap Screw:9
- Mate:18: Tetrix Flat 288mm x26mm(2):2 ↔ REV Expansion Hub:1
- Insert:286: REV Expansion Hub:1 ↔ Tetrix Screw 6-32 x 0.5(2):69
- Insert:287: REV Expansion Hub:1 ↔ Tetrix Screw 6-32 x 0.5(2):68
- Insert:288: Tetrix Flat 288mm x26mm(2):2 ↔ Tetrix Kep Nut(2):70
- Insert:289: Tetrix Flat 288mm x26mm(2):1 ↔ Tetrix Kep Nut(2):71
- Mate:19: Tetrix Inside C Connectors(2):4 ↔ Tetrix Screw 6-32 x 0.5(2):70
- Mate:20: Tetrix Inside C Connectors(2):4 ↔ Tetrix Screw 6-32 x 0.5(2):71
- Mate:21: Tetrix Flat 288mm x26mm(2):1 ↔ Tetrix Kep Nut(2):72
- Mate:22: Tetrix Flat 288mm x26mm(2):1 ↔ Tetrix Kep Nut(2):73
